# Autodesk Inventor assembly: Base
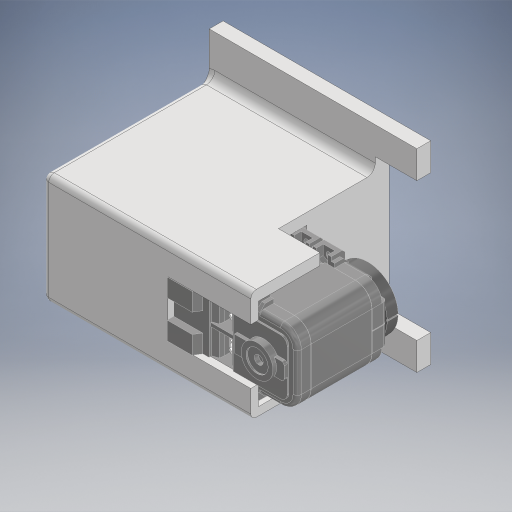
[picture p0: Inventor's stored thumbnail of the model, 512x512]
Saved by Autodesk Inventor 2024 (Build 280153000, 153)
## iProperties
Created: 2023-09-03
Part Number: Base
Document SubType Name: Assembly
Designer: arrusr01
Author: arrusr01
## Documents named in this file (3)
- C:\Users\arrusr01\OneDrive\Semestres\Inventor\Adaptable\Base.iam
- C:\Users\arrusr01\OneDrive\Semestres\Inventor\Adaptable\Base.ipt
- C:\Users\arrusr01\OneDrive\Semestres\Inventor\Adaptable\AX-12\AX-12.ipt
## Components (2 placed, 2 different names)
1. Base:1 — Mate:1, Mate:2, Mate:3
2. AX-12:1 — Mate:1, Mate:2, Mate:3
## Relationships (3: Mate 3)
- Mate:1: Base:1 ↔ AX-12:1
- Mate:2: Base:1 ↔ AX-12:1
- Mate:3: Base:1 ↔ AX-12:1
